# Autodesk Inventor assembly: GP4-100
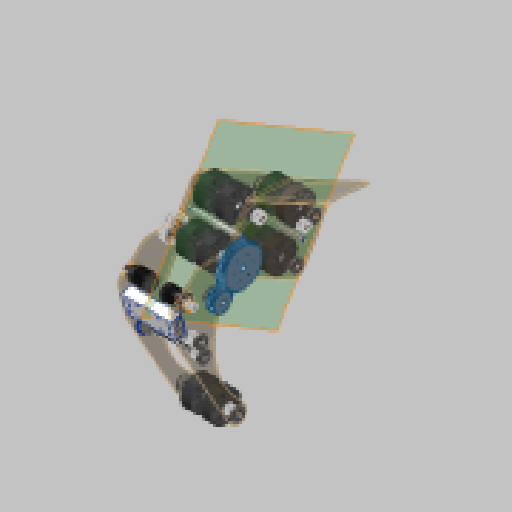
[picture p0: Inventor's stored thumbnail of the model, 512x512]
Saved by Autodesk Inventor 2023.5 (Build 275446000, 446)
## iProperties
Created: 2025-01-28
Part Number: GP4-100
Document SubType Name: Assembly
Designer: slick
Mass: 3702.68 g
Surface Area: 8972.54 cm^2
Volume: 1978.84 cm^3
Density: 1.87114 g/cm^3
Author: slick
## Documents named in this file (20)
- C:\Users\slick\OneDrive\Desktop\2025-ReefScape---CAD\Gripper\GP4\GP4-100.iam
- C:\Users\slick\OneDrive\Desktop\2025-ReefScape---CAD\Gripper\GP4\GP4-001.ipt
- C:\Users\slick\OneDrive\Desktop\2025-ReefScape---CAD\Gripper\GP4\GP4-002.ipt
- C:\Users\slick\OneDrive\Desktop\2025-ReefScape---CAD\Gripper\GP4\GP4-003.ipt
- C:\Users\slick\OneDrive\Desktop\2025-ReefScape---CAD\Gripper\GP4\GP4-003_MIR.ipt
- C:\Users\slick\OneDrive\Desktop\2025-ReefScape---CAD\COMMON PARTS\WHEELS\am-3945 3IN 500Hex Compliant Wheel REV 3.ipt
- C:\Users\slick\OneDrive\Desktop\2025-ReefScape---CAD\Gripper\GP4\GP4-005.ipt
- C:\Users\slick\OneDrive\Desktop\2025-ReefScape---CAD\Gripper\GP4\GP4-006.ipt
- C:\Users\slick\OneDrive\Desktop\2025-ReefScape---CAD\Gripper\GP4\GP4-007.ipt
- C:\Users\slick\OneDrive\Desktop\2025-ReefScape---CAD\COMMON PARTS\MOTORS\Minion.ipt
- C:\Users\slick\OneDrive\Desktop\2025-ReefScape---CAD\COMMON PARTS\PULLEYS\gt2\16T Gt2 Kracken PullyWCP-1178.ipt
- C:\Users\slick\OneDrive\Desktop\2025-ReefScape---CAD\COMMON PARTS\BEARINGS\13_75mm_1_2_ThunderHex_ID_x_1_125_OD_x_0_313_WD_Flanged_Bearing_217-4006_MIR.ipt
- C:\Users\slick\OneDrive\Desktop\2025-ReefScape---CAD\Gripper\GP4\GP4-008.ipt
- C:\Users\slick\OneDrive\Desktop\2025-ReefScape---CAD\COMMON PARTS\PULLEYS\gt2\60t_x_9mm_Wide_Double_Flange_Aluminum_Pulley_GT2_3mm_1_2_Hex_Bore_217-5876.ipt
- C:\Users\slick\OneDrive\Desktop\2025-ReefScape---CAD\COMMON PARTS\PULLEYS\gt2\24t_x_9mm_Wide_Double_Flange_Aluminum_Pulley_GT2_3mm_1_2_Hex_Bore_217-5875.ipt
- C:\Users\slick\OneDrive\Desktop\2025-ReefScape---CAD\COMMON PARTS\GEARS\20dp .5 hex\30t_Aluminum_Spur_Gear_20_DP_1_2_Hex_Bore_217-2705.ipt
- C:\Users\slick\OneDrive\Desktop\2025-ReefScape---CAD\Gripper\GP4\GP4-009.ipt
- C:\Users\slick\OneDrive\Desktop\2025-ReefScape---CAD\Gripper\GP4\GP4-010.ipt
- C:\Users\slick\OneDrive\Desktop\2025-ReefScape---CAD\COMMON PARTS\GEARS\Herringbone\herringbone 2m 24t\herringbone 2m 24t.ipt
- C:\Users\slick\OneDrive\Desktop\2025-ReefScape---CAD\COMMON PARTS\GEARS\Herringbone\2m 36t herringbone\2m 36t herringbone.ipt
## Components (55 placed, 19 different names)
1. GP4-008:1 — Insert:1, Insert:2, Mate:2, Mate:6, Mate:11, Insert:21, Insert:26, Insert:27, Insert:28, Mate:41, Mate:42, Insert:29, Insert:30
2. GP4-002:1 — Flush:1, Flush:2, Flush:3, Mate:1, Flush:4, Flush:5
3. GP4-003:1 — Flush:1, Mate:1, Flush:4, Insert:1, Insert:2
4. GP4-003_MIR:1 — Flush:2, Flush:3, Flush:5, Insert:3, Insert:4
5. GP4-001:2 — Insert:3, Insert:4, Mate:7, Mate:10, Mate:12, Mate:23, Mate:24, Insert:7, Insert:14, Insert:15, Insert:16, Mate:27, Insert:19
6. GP4-006:1 — Mate:12, Mate:20, Mate:21, Mate:22, Symmetry:1, Insert:11, Insert:12, Insert:13, Mate:27, Insert:17, Insert:18, Insert:20, Insert:32
7. GP4-005:2 — Mate:11, Mate:15, Mate:22, Symmetry:1, Insert:5, Insert:6, Insert:22, Insert:23, Insert:24, Insert:25, Insert:33, Insert:34
8. GP4-007:1 — Insert:6, Insert:18
9. GP4-007:2 — Insert:5, Insert:17
10. Minion:1 — Mate:23, Mate:24, Insert:7, Mate:25, Flush:11
11. 16T Gt2 Kracken PullyWCP-1178:1 — Mate:25, Flush:11, Flush:15
12. 60t_x_9mm_Wide_Double_Flange_Aluminum_Pulley_GT2_3mm_1_2_Hex_Bore_217-5876:1 — Mate:28, Flush:15
13. 24t_x_9mm_Wide_Double_Flange_Aluminum_Pulley_GT2_3mm_1_2_Hex_Bore_217-5875:1 — Mate:32, Flush:14
14. 24t_x_9mm_Wide_Double_Flange_Aluminum_Pulley_GT2_3mm_1_2_Hex_Bore_217-5875:2 — Mate:31, Flush:13, Flush:14
15. 24t_x_9mm_Wide_Double_Flange_Aluminum_Pulley_GT2_3mm_1_2_Hex_Bore_217-5875:3 — Mate:30, Flush:13, Flush:17
16. 24t_x_9mm_Wide_Double_Flange_Aluminum_Pulley_GT2_3mm_1_2_Hex_Bore_217-5875:4 — Mate:29, Mate:37, Flush:17
17. 30t_Aluminum_Spur_Gear_20_DP_1_2_Hex_Bore_217-2705:1 — Mate:34, Flush:16, Mate:36, Mate:39, Flush:19
18. 30t_Aluminum_Spur_Gear_20_DP_1_2_Hex_Bore_217-2705:2 — Mate:35, Flush:16, Mate:38, Flush:18
19. GP4-009:1 — Mate:38, Flush:18
20. GP4-009:2 — Mate:39, Flush:19
21. GP4-010:1 — Mate:40, Flush:20
22. Minion:2 — Mate:41, Mate:42, Insert:29, Mate:43, Flush:21
23. 16T Gt2 Kracken PullyWCP-1178:2 — Mate:43, Flush:21
24. herringbone 2m 24t:1 — Mate:44, Flush:22, Rotation:1
25. 24t_x_9mm_Wide_Double_Flange_Aluminum_Pulley_GT2_3mm_1_2_Hex_Bore_217-5875:5 — Mate:46
26. 24t_x_9mm_Wide_Double_Flange_Aluminum_Pulley_GT2_3mm_1_2_Hex_Bore_217-5875:6 — Mate:47
27. 2m 36t herringbone:1 — Insert:33, Insert:34, Flush:22, Rotation:1
28. am-3945 3IN 500Hex Compliant Wheel REV 3:10
29. am-3945 3IN 500Hex Compliant Wheel REV 3:9 — Mate:21, Flush:9
30. am-3945 3IN 500Hex Compliant Wheel REV 3:8
31. am-3945 3IN 500Hex Compliant Wheel REV 3:7 — Mate:20, Flush:10
32. am-3945 3IN 500Hex Compliant Wheel REV 3:6 — Mate:2, Mate:3, Flush:6, Flush:9
33. am-3945 3IN 500Hex Compliant Wheel REV 3:5 — Mate:3, Flush:7, Mate:10
34. am-3945 3IN 500Hex Compliant Wheel REV 3:4 — Mate:6, Mate:8
35. am-3945 3IN 500Hex Compliant Wheel REV 3:3 — Mate:7, Mate:8, Flush:8
36. am-3945 3IN 500Hex Compliant Wheel REV 3:2 — Mate:5, Mate:9, Flush:7, Flush:8
37. am-3945 3IN 500Hex Compliant Wheel REV 3:1 — Mate:5, Mate:9, Flush:6, Mate:15, Flush:10
38. 13_75mm_1_2_ThunderHex_ID_x_1_125_OD_x_0_313_WD_Flanged_Bearing_217-4006_MIR:19 — Insert:32, Mate:47
39. 13_75mm_1_2_ThunderHex_ID_x_1_125_OD_x_0_313_WD_Flanged_Bearing_217-4006_MIR:18 — Insert:30, Mate:44
40. 13_75mm_1_2_ThunderHex_ID_x_1_125_OD_x_0_313_WD_Flanged_Bearing_217-4006_MIR:10 — Insert:21
41. 13_75mm_1_2_ThunderHex_ID_x_1_125_OD_x_0_313_WD_Flanged_Bearing_217-4006_MIR:11 — Insert:22
42. 13_75mm_1_2_ThunderHex_ID_x_1_125_OD_x_0_313_WD_Flanged_Bearing_217-4006_MIR:12 — Insert:23
43. 13_75mm_1_2_ThunderHex_ID_x_1_125_OD_x_0_313_WD_Flanged_Bearing_217-4006_MIR:13 — Insert:24
44. 13_75mm_1_2_ThunderHex_ID_x_1_125_OD_x_0_313_WD_Flanged_Bearing_217-4006_MIR:14 — Insert:25
45. 13_75mm_1_2_ThunderHex_ID_x_1_125_OD_x_0_313_WD_Flanged_Bearing_217-4006_MIR:15 — Insert:28
46. 13_75mm_1_2_ThunderHex_ID_x_1_125_OD_x_0_313_WD_Flanged_Bearing_217-4006_MIR:16 — Insert:27
47. 13_75mm_1_2_ThunderHex_ID_x_1_125_OD_x_0_313_WD_Flanged_Bearing_217-4006_MIR:17 — Insert:26, Mate:37
48. 13_75mm_1_2_ThunderHex_ID_x_1_125_OD_x_0_313_WD_Flanged_Bearing_217-4006_MIR:1 — Insert:15, Mate:30, Mate:35
49. 13_75mm_1_2_ThunderHex_ID_x_1_125_OD_x_0_313_WD_Flanged_Bearing_217-4006_MIR:3 — Insert:20, Mate:32
50. 13_75mm_1_2_ThunderHex_ID_x_1_125_OD_x_0_313_WD_Flanged_Bearing_217-4006_MIR:4 — Insert:14, Mate:31, Mate:34, Mate:36
51. 13_75mm_1_2_ThunderHex_ID_x_1_125_OD_x_0_313_WD_Flanged_Bearing_217-4006_MIR:5 — Insert:13
52. 13_75mm_1_2_ThunderHex_ID_x_1_125_OD_x_0_313_WD_Flanged_Bearing_217-4006_MIR:6 — Insert:12
53. 13_75mm_1_2_ThunderHex_ID_x_1_125_OD_x_0_313_WD_Flanged_Bearing_217-4006_MIR:7 — Insert:11, Mate:46
54. 13_75mm_1_2_ThunderHex_ID_x_1_125_OD_x_0_313_WD_Flanged_Bearing_217-4006_MIR:8 — Insert:19, Mate:28
55. 13_75mm_1_2_ThunderHex_ID_x_1_125_OD_x_0_313_WD_Flanged_Bearing_217-4006_MIR:9 — Insert:16, Mate:29, Mate:40, Flush:20
## Relationships (94: Mate 41, Insert 30, Flush 21, Symmetry 1, RelateRotation 1)
- Flush:1: GP4-002:1 ↔ GP4-003:1
- Flush:2: GP4-002:1 ↔ GP4-003_MIR:1
- Flush:3: GP4-002:1 ↔ GP4-003_MIR:1
- Mate:1: GP4-002:1 ↔ GP4-003:1
- Flush:4: GP4-002:1 ↔ GP4-003:1
- Flush:5: GP4-002:1 ↔ GP4-003_MIR:1
- Insert:1: GP4-008:1 ↔ GP4-003:1
- Insert:2: GP4-008:1 ↔ GP4-003:1
- Insert:3: GP4-003_MIR:1 ↔ GP4-001:2
- Insert:4: GP4-003_MIR:1 ↔ GP4-001:2
- Mate:2: GP4-008:1 ↔ am-3945 3IN 500Hex Compliant Wheel REV 3:6
- Mate:3: am-3945 3IN 500Hex Compliant Wheel REV 3:6 ↔ am-3945 3IN 500Hex Compliant Wheel REV 3:5
- Mate:5: am-3945 3IN 500Hex Compliant Wheel REV 3:2 ↔ am-3945 3IN 500Hex Compliant Wheel REV 3:1
- Mate:6: GP4-008:1 ↔ am-3945 3IN 500Hex Compliant Wheel REV 3:4
- Mate:7: GP4-001:2 ↔ am-3945 3IN 500Hex Compliant Wheel REV 3:3
- Mate:8 (25.4 mm): am-3945 3IN 500Hex Compliant Wheel REV 3:4 ↔ am-3945 3IN 500Hex Compliant Wheel REV 3:3
- Mate:9 (25.4 mm): am-3945 3IN 500Hex Compliant Wheel REV 3:2 ↔ am-3945 3IN 500Hex Compliant Wheel REV 3:1
- Flush:6: am-3945 3IN 500Hex Compliant Wheel REV 3:6 ↔ am-3945 3IN 500Hex Compliant Wheel REV 3:1
- Flush:7: am-3945 3IN 500Hex Compliant Wheel REV 3:5 ↔ am-3945 3IN 500Hex Compliant Wheel REV 3:2
- Mate:10 (25.4 mm): GP4-001:2 ↔ am-3945 3IN 500Hex Compliant Wheel REV 3:5
- Flush:8: am-3945 3IN 500Hex Compliant Wheel REV 3:3 ↔ am-3945 3IN 500Hex Compliant Wheel REV 3:2
- Mate:11: GP4-008:1 ↔ GP4-005:2
- Mate:12: GP4-001:2 ↔ GP4-006:1
- Mate:15: GP4-005:2 ↔ am-3945 3IN 500Hex Compliant Wheel REV 3:1
- [Mate]: am-3945 3IN 500Hex Compliant Wheel REV 3:8 ↔ am-3945 3IN 500Hex Compliant Wheel REV 3:7
- [Mate] (25.4 mm): am-3945 3IN 500Hex Compliant Wheel REV 3:8 ↔ am-3945 3IN 500Hex Compliant Wheel REV 3:7
- [Mate]: am-3945 3IN 500Hex Compliant Wheel REV 3:10 ↔ am-3945 3IN 500Hex Compliant Wheel REV 3:9
- [Mate] (25.4 mm): am-3945 3IN 500Hex Compliant Wheel REV 3:10 ↔ am-3945 3IN 500Hex Compliant Wheel REV 3:9
- Mate:20: GP4-006:1 ↔ am-3945 3IN 500Hex Compliant Wheel REV 3:7
- Mate:21: GP4-006:1 ↔ am-3945 3IN 500Hex Compliant Wheel REV 3:9
- Flush:9: am-3945 3IN 500Hex Compliant Wheel REV 3:9 ↔ am-3945 3IN 500Hex Compliant Wheel REV 3:6
- Flush:10: am-3945 3IN 500Hex Compliant Wheel REV 3:7 ↔ am-3945 3IN 500Hex Compliant Wheel REV 3:1
- Mate:22: GP4-006:1 ↔ GP4-005:2
- Symmetry:1: GP4-006:1 ↔ GP4-005:2
- Insert:5: GP4-005:2 ↔ GP4-007:2
- Insert:6: GP4-005:2 ↔ GP4-007:1
- Mate:23: GP4-001:2 ↔ Minion:1
- Mate:24: GP4-001:2 ↔ Minion:1
- Insert:7: GP4-001:2 ↔ Minion:1
- Mate:25: Minion:1 ↔ 16T Gt2 Kracken PullyWCP-1178:1
- Flush:11: Minion:1 ↔ 16T Gt2 Kracken PullyWCP-1178:1
- Insert:11: GP4-006:1 ↔ 13_75mm_1_2_ThunderHex_ID_x_1_125_OD_x_0_313_WD_Flanged_Bearing_217-4006_MIR:7
- Insert:12: GP4-006:1 ↔ 13_75mm_1_2_ThunderHex_ID_x_1_125_OD_x_0_313_WD_Flanged_Bearing_217-4006_MIR:6
- Insert:13: GP4-006:1 ↔ 13_75mm_1_2_ThunderHex_ID_x_1_125_OD_x_0_313_WD_Flanged_Bearing_217-4006_MIR:5
- Insert:14: GP4-001:2 ↔ 13_75mm_1_2_ThunderHex_ID_x_1_125_OD_x_0_313_WD_Flanged_Bearing_217-4006_MIR:4
- Insert:15: GP4-001:2 ↔ 13_75mm_1_2_ThunderHex_ID_x_1_125_OD_x_0_313_WD_Flanged_Bearing_217-4006_MIR:1
- Insert:16: GP4-001:2 ↔ 13_75mm_1_2_ThunderHex_ID_x_1_125_OD_x_0_313_WD_Flanged_Bearing_217-4006_MIR:9
- Mate:27: GP4-001:2 ↔ GP4-006:1
- Insert:17: GP4-006:1 ↔ GP4-007:2
- Insert:18: GP4-006:1 ↔ GP4-007:1
- Insert:19: GP4-001:2 ↔ 13_75mm_1_2_ThunderHex_ID_x_1_125_OD_x_0_313_WD_Flanged_Bearing_217-4006_MIR:8
- Insert:20: GP4-006:1 ↔ 13_75mm_1_2_ThunderHex_ID_x_1_125_OD_x_0_313_WD_Flanged_Bearing_217-4006_MIR:3
- Mate:28: 60t_x_9mm_Wide_Double_Flange_Aluminum_Pulley_GT2_3mm_1_2_Hex_Bore_217-5876:1 ↔ 13_75mm_1_2_ThunderHex_ID_x_1_125_OD_x_0_313_WD_Flanged_Bearing_217-4006_MIR:8
- Mate:29: 24t_x_9mm_Wide_Double_Flange_Aluminum_Pulley_GT2_3mm_1_2_Hex_Bore_217-5875:4 ↔ 13_75mm_1_2_ThunderHex_ID_x_1_125_OD_x_0_313_WD_Flanged_Bearing_217-4006_MIR:9
- Mate:30: 24t_x_9mm_Wide_Double_Flange_Aluminum_Pulley_GT2_3mm_1_2_Hex_Bore_217-5875:3 ↔ 13_75mm_1_2_ThunderHex_ID_x_1_125_OD_x_0_313_WD_Flanged_Bearing_217-4006_MIR:1
- Mate:31: 24t_x_9mm_Wide_Double_Flange_Aluminum_Pulley_GT2_3mm_1_2_Hex_Bore_217-5875:2 ↔ 13_75mm_1_2_ThunderHex_ID_x_1_125_OD_x_0_313_WD_Flanged_Bearing_217-4006_MIR:4
- Mate:32: 24t_x_9mm_Wide_Double_Flange_Aluminum_Pulley_GT2_3mm_1_2_Hex_Bore_217-5875:1 ↔ 13_75mm_1_2_ThunderHex_ID_x_1_125_OD_x_0_313_WD_Flanged_Bearing_217-4006_MIR:3
- Flush:13: 24t_x_9mm_Wide_Double_Flange_Aluminum_Pulley_GT2_3mm_1_2_Hex_Bore_217-5875:2 ↔ 24t_x_9mm_Wide_Double_Flange_Aluminum_Pulley_GT2_3mm_1_2_Hex_Bore_217-5875:3
- Flush:14: 24t_x_9mm_Wide_Double_Flange_Aluminum_Pulley_GT2_3mm_1_2_Hex_Bore_217-5875:1 ↔ 24t_x_9mm_Wide_Double_Flange_Aluminum_Pulley_GT2_3mm_1_2_Hex_Bore_217-5875:2
- Flush:15: 16T Gt2 Kracken PullyWCP-1178:1 ↔ 60t_x_9mm_Wide_Double_Flange_Aluminum_Pulley_GT2_3mm_1_2_Hex_Bore_217-5876:1
- Mate:34: 30t_Aluminum_Spur_Gear_20_DP_1_2_Hex_Bore_217-2705:1 ↔ 13_75mm_1_2_ThunderHex_ID_x_1_125_OD_x_0_313_WD_Flanged_Bearing_217-4006_MIR:4
- Mate:35: 30t_Aluminum_Spur_Gear_20_DP_1_2_Hex_Bore_217-2705:2 ↔ 13_75mm_1_2_ThunderHex_ID_x_1_125_OD_x_0_313_WD_Flanged_Bearing_217-4006_MIR:1
- Flush:16: 30t_Aluminum_Spur_Gear_20_DP_1_2_Hex_Bore_217-2705:1 ↔ 30t_Aluminum_Spur_Gear_20_DP_1_2_Hex_Bore_217-2705:2
- Mate:36 (3.175 mm): 30t_Aluminum_Spur_Gear_20_DP_1_2_Hex_Bore_217-2705:1 ↔ 13_75mm_1_2_ThunderHex_ID_x_1_125_OD_x_0_313_WD_Flanged_Bearing_217-4006_MIR:4
- Insert:21: GP4-008:1 ↔ 13_75mm_1_2_ThunderHex_ID_x_1_125_OD_x_0_313_WD_Flanged_Bearing_217-4006_MIR:10
- Insert:22: GP4-005:2 ↔ 13_75mm_1_2_ThunderHex_ID_x_1_125_OD_x_0_313_WD_Flanged_Bearing_217-4006_MIR:11
- Insert:23: GP4-005:2 ↔ 13_75mm_1_2_ThunderHex_ID_x_1_125_OD_x_0_313_WD_Flanged_Bearing_217-4006_MIR:12
- Insert:24: GP4-005:2 ↔ 13_75mm_1_2_ThunderHex_ID_x_1_125_OD_x_0_313_WD_Flanged_Bearing_217-4006_MIR:13
- Insert:25: GP4-005:2 ↔ 13_75mm_1_2_ThunderHex_ID_x_1_125_OD_x_0_313_WD_Flanged_Bearing_217-4006_MIR:14
- Insert:26: GP4-008:1 ↔ 13_75mm_1_2_ThunderHex_ID_x_1_125_OD_x_0_313_WD_Flanged_Bearing_217-4006_MIR:17
- Insert:27: GP4-008:1 ↔ 13_75mm_1_2_ThunderHex_ID_x_1_125_OD_x_0_313_WD_Flanged_Bearing_217-4006_MIR:16
- Insert:28: GP4-008:1 ↔ 13_75mm_1_2_ThunderHex_ID_x_1_125_OD_x_0_313_WD_Flanged_Bearing_217-4006_MIR:15
- Mate:37 (3.175 mm): 24t_x_9mm_Wide_Double_Flange_Aluminum_Pulley_GT2_3mm_1_2_Hex_Bore_217-5875:4 ↔ 13_75mm_1_2_ThunderHex_ID_x_1_125_OD_x_0_313_WD_Flanged_Bearing_217-4006_MIR:17
- Flush:17: 24t_x_9mm_Wide_Double_Flange_Aluminum_Pulley_GT2_3mm_1_2_Hex_Bore_217-5875:3 ↔ 24t_x_9mm_Wide_Double_Flange_Aluminum_Pulley_GT2_3mm_1_2_Hex_Bore_217-5875:4
- Mate:38: 30t_Aluminum_Spur_Gear_20_DP_1_2_Hex_Bore_217-2705:2 ↔ GP4-009:1
- Mate:39: 30t_Aluminum_Spur_Gear_20_DP_1_2_Hex_Bore_217-2705:1 ↔ GP4-009:2
- Flush:18: 30t_Aluminum_Spur_Gear_20_DP_1_2_Hex_Bore_217-2705:2 ↔ GP4-009:1
- Flush:19: 30t_Aluminum_Spur_Gear_20_DP_1_2_Hex_Bore_217-2705:1 ↔ GP4-009:2
- Mate:40: GP4-010:1 ↔ 13_75mm_1_2_ThunderHex_ID_x_1_125_OD_x_0_313_WD_Flanged_Bearing_217-4006_MIR:9
- Flush:20: GP4-010:1 ↔ 13_75mm_1_2_ThunderHex_ID_x_1_125_OD_x_0_313_WD_Flanged_Bearing_217-4006_MIR:9
- Mate:41: GP4-008:1 ↔ Minion:2
- Mate:42: GP4-008:1 ↔ Minion:2
- Insert:29: GP4-008:1 ↔ Minion:2
- Mate:43: Minion:2 ↔ 16T Gt2 Kracken PullyWCP-1178:2
- Flush:21: Minion:2 ↔ 16T Gt2 Kracken PullyWCP-1178:2
- Insert:30: GP4-008:1 ↔ 13_75mm_1_2_ThunderHex_ID_x_1_125_OD_x_0_313_WD_Flanged_Bearing_217-4006_MIR:18
- Mate:44: herringbone 2m 24t:1 ↔ 13_75mm_1_2_ThunderHex_ID_x_1_125_OD_x_0_313_WD_Flanged_Bearing_217-4006_MIR:18
- Insert:32: GP4-006:1 ↔ 13_75mm_1_2_ThunderHex_ID_x_1_125_OD_x_0_313_WD_Flanged_Bearing_217-4006_MIR:19
- Mate:46: 24t_x_9mm_Wide_Double_Flange_Aluminum_Pulley_GT2_3mm_1_2_Hex_Bore_217-5875:5 ↔ 13_75mm_1_2_ThunderHex_ID_x_1_125_OD_x_0_313_WD_Flanged_Bearing_217-4006_MIR:7
- Mate:47: 24t_x_9mm_Wide_Double_Flange_Aluminum_Pulley_GT2_3mm_1_2_Hex_Bore_217-5875:6 ↔ 13_75mm_1_2_ThunderHex_ID_x_1_125_OD_x_0_313_WD_Flanged_Bearing_217-4006_MIR:19
- Insert:33: GP4-005:2 ↔ 2m 36t herringbone:1
- Insert:34: GP4-005:2 ↔ 2m 36t herringbone:1
- Flush:22: herringbone 2m 24t:1 ↔ 2m 36t herringbone:1
- Rotation:1 [RelateRotation] (1 ul): herringbone 2m 24t:1 ↔ 2m 36t herringbone:1
## Named parameters: d53_d33 = 0 mm, d54_d37 = 25.4 mm, d55_d33 = 0 mm, d56_d37 = 25.4 mm
